# Autodesk Inventor assembly: ensamble
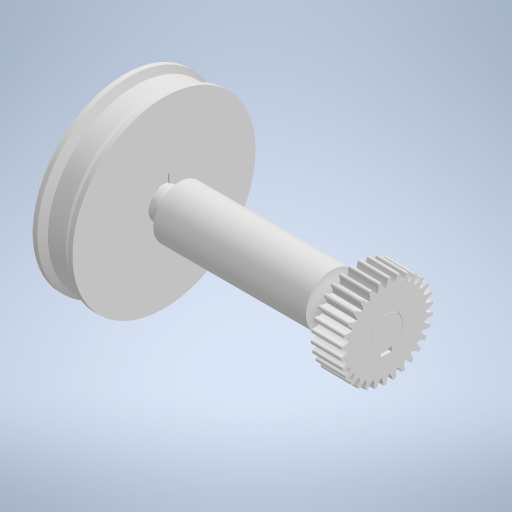
[picture p0: Inventor's stored thumbnail of the model, 512x512]
Saved by Autodesk Inventor 2024 (Build 280153000, 153)
## iProperties
Created: 2024-03-30
Part Number: ensamble
Document SubType Name: Assembly
Designer: JavierJ
Author: JavierJ
## Documents named in this file (5)
- C:\Users\JavierJ\Documents\Javier\SEMESTRE 1 2024\LAB DINAMICA\ensamble.iam
- C:\Users\JavierJ\Downloads\POLEA.ipt
- C:\Users\JavierJ\Downloads\ENGRANE.ipt
- C:\Users\JavierJ\Downloads\CUÑA.ipt
- C:\Users\JavierJ\Downloads\EJE_CUÑEROS.ipt
## Components (5 placed, 4 different names)
1. POLEA:1 — Rigid:3
2. ENGRANE:1
3. CUÑA:1 — Rigid:2, Rigid:3
4. CUÑA:2 — Tangent:1, Tangent:2, Rigid:1
5. EJE_CUÑEROS:1 — Tangent:1, Tangent:2, Rigid:1, Rigid:2
## Relationships (5: WeldJoint 3, Tangent 2)
- Tangent:1: CUÑA:2 ↔ EJE_CUÑEROS:1
- Tangent:2: CUÑA:2 ↔ EJE_CUÑEROS:1
- Rigid:1 [WeldJoint]: CUÑA:2 ↔ EJE_CUÑEROS:1
- Rigid:2 [WeldJoint]: CUÑA:1 ↔ EJE_CUÑEROS:1
- Rigid:3 [WeldJoint]: POLEA:1 ↔ CUÑA:1
